# Autodesk Inventor assembly: CE-7.1.1_MB
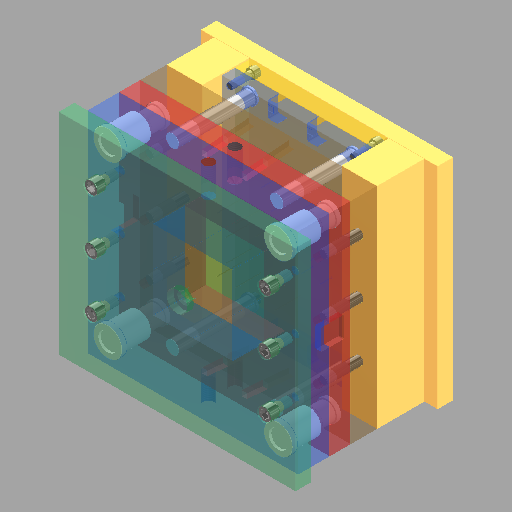
[picture p0: Inventor's stored thumbnail of the model, 512x512]
Saved by Autodesk Inventor 2024 (Build 280153000, 153)
## iProperties
Created: 2024-02-25
Part Number: CE-7.1.1_MB
Document SubType Name: Assembly
Designer: Alex
Author: Alex
## Documents named in this file (16)
- C:\Shared\alex-bartella-schoolwork\4z03\Week 6\MB\FUTABA_SA-S 1\CE-7.1.1_MB.iam
- C:\Users\turbo\Documents\Inventor\Content Center Files\R2024\en-US\JIS 1176\JIS 1176 M12x40.ipt
- C:\Users\turbo\Documents\Inventor\Content Center Files\R2024\en-US\GBA\M-GBA 35x59.ipt
- C:\Shared\alex-bartella-schoolwork\4z03\Week 6\MB\FUTABA_SA-S 1\CE-7.1.1_MB_SA-SB1.ipt
- C:\Shared\alex-bartella-schoolwork\4z03\Week 6\MB\FUTABA_SA-S 1\CE-7.1.1_MB_SA-SB2.ipt
- C:\Shared\alex-bartella-schoolwork\4z03\Week 6\MB\FUTABA_SA-S 1\CE-7.1.1_MB_SA-EP.ipt
- C:\Users\turbo\Documents\Inventor\Content Center Files\R2024\en-US\GPA\M-GPA35x97x39.ipt
- C:\Shared\alex-bartella-schoolwork\4z03\Week 6\MB\FUTABA_SA-S 1\CE-7.1.1_MB_SA-ERP.ipt
- C:\Shared\alex-bartella-schoolwork\4z03\Week 6\MB\FUTABA_SA-S 1\CE-7.1.1_MB_SA-BCP.ipt
- C:\Users\turbo\Documents\Inventor\Content Center Files\R2024\en-US\JIS 1176\JIS 1176 M16x30.ipt
- C:\Shared\alex-bartella-schoolwork\4z03\Week 6\MB\FUTABA_SA-S 1\CE-7.1.1_MB_RPN.ipt
- C:\Shared\alex-bartella-schoolwork\4z03\Week 6\MB\FUTABA_SA-S 1\CE-7.1.1_MB_SA-S-AP.ipt
- C:\Shared\alex-bartella-schoolwork\4z03\Week 6\MB\FUTABA_SA-S 1\CE-7.1.1_MB_SA-S-BP.ipt
- C:\Shared\alex-bartella-schoolwork\4z03\Week 6\MB\FUTABA_SA-S 1\CE-7.1.1_MB_SA-TCP.ipt
- C:\Shared\alex-bartella-schoolwork\4z03\Week 6\MB\FUTABA_SA-S 1\CE-7.1.1_MB_SA-SP.ipt
- C:\Users\turbo\Documents\Inventor\Content Center Files\R2024\en-US\JIS 1176\JIS 1176 M16x170.ipt
## Components (37 placed, 15 different names)
1. CE-7.1.1_MB_SA-SB1:1 — Flush:1, Flush:3, Mate:1, Mate:5
2. CE-7.1.1_MB_SA-SB2:2 — Flush:2, Flush:4, Mate:2, Mate:6
3. CE-7.1.1_MB_SA-EP:1 — Insert:1, Flush:5, Flush:6, Ejection, Mate:4
4. CE-7.1.1_MB_SA-ERP:1 — Insert:7, Flush:7, Flush:8, Mate:4
5. CE-7.1.1_MB_SA-BCP:1 — Insert:8, Ejection, Flush:9, Flush:10, Mate:5, Mate:6
6. CE-7.1.1_MB_SA-S-AP:1 — Insert:2, Insert:5, Flush:11, Flush:12, Mate:7, PL1, Flush:19
7. CE-7.1.1_MB_SA-S-BP:1 — Insert:3, Insert:4, Flush:13, Flush:14, PL1, Mate:9
8. CE-7.1.1_MB_SA-TCP:1 — Insert:6, Mate:7, Flush:15, Flush:16
9. CE-7.1.1_MB_SA-SP:1 — Mate:1, Mate:2, Flush:17, Flush:18, Mate:9
10. GPA 35x97x39:1 — Insert:3
11. GPA 35x97x39:3
12. JIS 1176 M16x30:1 — Insert:6
13. JIS 1176 M16x30:2
14. JIS 1176 M16x30:3
15. JIS 1176 M16x30:4
16. JIS 1176 M16x30:5
17. JIS 1176 M16x30:6
18. JIS 1176 M12x40:1 — Insert:1
19. JIS 1176 M12x40:2
20. JIS 1176 M12x40:3
21. JIS 1176 M12x40:4
22. JIS 1176 M16x170:1 — Insert:8
23. JIS 1176 M16x170:2
24. JIS 1176 M16x170:3
25. JIS 1176 M16x170:4
26. JIS 1176 M16x170:5
27. JIS 1176 M16x170:6
28. GBA 35x59:1 — Insert:2
29. GBA 35x59:3
30. GPA 35x97x39:2 — Insert:4
31. GPA 35x97x39:4
32. CE-7.1.1_MB_RPN:1 — Insert:7
33. CE-7.1.1_MB_RPN:2
34. CE-7.1.1_MB_RPN:3
35. CE-7.1.1_MB_RPN:4
36. GBA 35x59:2 — Insert:5
37. GBA 35x59:4
## Component patterns: (2 elements, first: GPA 35x97x39:1), (6 elements, first: JIS 1176 M16x30:1), (4 elements, first: JIS 1176 M12x40:1), (6 elements, first: JIS 1176 M16x170:1), (2 elements, first: GBA 35x59:1), (2 elements, first: GPA 35x97x39:2), (4 elements, first: CE-7.1.1_MB_RPN:1), (2 elements, first: GBA 35x59:2)
## Relationships (36: Flush 19, Mate 9, Insert 8)
- Insert:1: CE-7.1.1_MB_SA-EP:1 ↔ JIS 1176 M12x40:1
- Insert:2: CE-7.1.1_MB_SA-S-AP:1 ↔ GBA 35x59:1
- Insert:3: CE-7.1.1_MB_SA-S-BP:1 ↔ GPA 35x97x39:1
- Insert:4: CE-7.1.1_MB_SA-S-BP:1 ↔ GPA 35x97x39:2
- Insert:5: CE-7.1.1_MB_SA-S-AP:1 ↔ GBA 35x59:2
- Insert:6: CE-7.1.1_MB_SA-TCP:1 ↔ JIS 1176 M16x30:1
- Insert:7: CE-7.1.1_MB_SA-ERP:1 ↔ CE-7.1.1_MB_RPN:1
- Insert:8: CE-7.1.1_MB_SA-BCP:1 ↔ JIS 1176 M16x170:1
- Flush:1: CE-7.1.1_MB_SA-SB1:1
- Flush:2: CE-7.1.1_MB_SA-SB2:2
- Flush:3: CE-7.1.1_MB_SA-SB1:1
- Flush:4: CE-7.1.1_MB_SA-SB2:2
- Mate:1: CE-7.1.1_MB_SA-SB1:1 ↔ CE-7.1.1_MB_SA-SP:1
- Mate:2: CE-7.1.1_MB_SA-SB2:2 ↔ CE-7.1.1_MB_SA-SP:1
- Flush:5: CE-7.1.1_MB_SA-EP:1
- Flush:6: CE-7.1.1_MB_SA-EP:1
- Ejection [Mate]: CE-7.1.1_MB_SA-EP:1 ↔ CE-7.1.1_MB_SA-BCP:1
- Flush:7: CE-7.1.1_MB_SA-ERP:1
- Flush:8: CE-7.1.1_MB_SA-ERP:1
- Mate:4: CE-7.1.1_MB_SA-EP:1 ↔ CE-7.1.1_MB_SA-ERP:1
- Flush:9: CE-7.1.1_MB_SA-BCP:1
- Flush:10: CE-7.1.1_MB_SA-BCP:1
- Mate:5: CE-7.1.1_MB_SA-SB1:1 ↔ CE-7.1.1_MB_SA-BCP:1
- Mate:6: CE-7.1.1_MB_SA-SB2:2 ↔ CE-7.1.1_MB_SA-BCP:1
- Flush:11: CE-7.1.1_MB_SA-S-AP:1
- Flush:12: CE-7.1.1_MB_SA-S-AP:1
- Mate:7: CE-7.1.1_MB_SA-S-AP:1 ↔ CE-7.1.1_MB_SA-TCP:1
- Flush:13: CE-7.1.1_MB_SA-S-BP:1
- Flush:14: CE-7.1.1_MB_SA-S-BP:1
- PL1 [Mate]: CE-7.1.1_MB_SA-S-AP:1 ↔ CE-7.1.1_MB_SA-S-BP:1
- Flush:15: CE-7.1.1_MB_SA-TCP:1
- Flush:16: CE-7.1.1_MB_SA-TCP:1
- Flush:17: CE-7.1.1_MB_SA-SP:1
- Flush:18: CE-7.1.1_MB_SA-SP:1
- Mate:9: CE-7.1.1_MB_SA-S-BP:1 ↔ CE-7.1.1_MB_SA-SP:1
- Flush:19: CE-7.1.1_MB_SA-S-AP:1
